# Autodesk Inventor assembly: Antriebsstrang
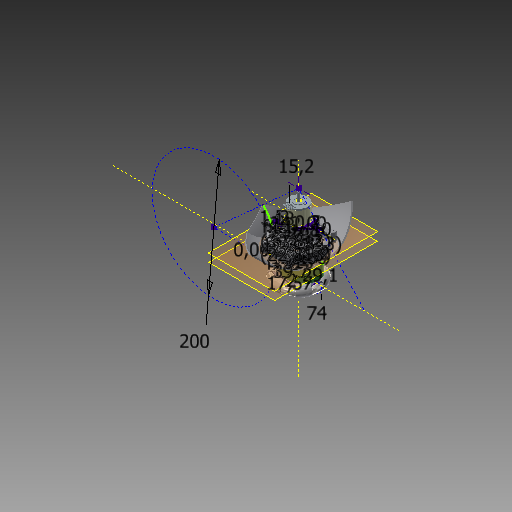
[picture p0: Inventor's stored thumbnail of the model, 512x512]
Saved by Autodesk Inventor 2018.3 (Build 223284000, 284)
## iProperties
Created: 2018-06-25
Part Number: Antriebsstrang
Material: Generisch
Document SubType Name: Assembly
Designer: JochenAlt
Author: JochenAlt
## Documents named in this file (15)
- D:\Projects\FlowerPot\CAD\DriveChain.iam
- D:\Projects\FlowerPot\CAD\OmniWheel.ipt
- D:\Projects\FlowerPot\CAD\Mounting Hub.ipt
- D:\Projects\FlowerPot\CAD\Encoder\Avago Encoder.iam
- D:\Projects\FlowerPot\CAD\HarmonicDrive-Axis.ipt
- C:\Users\JochenAlt\Documents\Inventor\Content Center Files\R2018\de-DE\AS 1420\AS 1420 - 1973 - M3 x 8.ipt
- C:\Users\JochenAlt\Documents\Inventor\Content Center Files\R2018\de-DE\DIN 912\DIN 912 - M2 x 0,4 x 8 x 7.ipt
- C:\Users\JochenAlt\Documents\Inventor\Content Center Files\R2018\de-DE\DIN 934\DIN 934 - M2 x 0,4.ipt
- D:\Projects\FlowerPot\CAD\BushOmniWheel.ipt
- C:\Users\JochenAlt\Documents\Inventor\Content Center Files\R2018\de-DE\DIN BEARING(1)\DIN 625 SKF - SKF 623.ipt
- D:\Projects\FlowerPot\CAD\Motor.iam
- D:\Projects\FlowerPot\CAD\PlanetaryGear\PlanetaryGear.iam
- D:\Projects\FlowerPot\CAD\BushingPlanetaryGearLeft.ipt
- D:\Projects\FlowerPot\CAD\DriveChainEnclosure.ipt
- D:\Projects\FlowerPot\CAD\EncoderBushRight.ipt
## Components (30 placed, 14 different names)
1. OmniWheel:1 — Passend:1, Passend:3, Passend:4, Passend:5, Passend:6, Passend:7, Passend:8, Passend:9, Passend:10, Passend:11, Passend:12, Passend:14, Passend:16, Passend:18, Passend:20, Passend:22, Passend:24
2. Mounting Hub:1 — Passend:1, Passend:25, Passend:30, Passend:31, Drehung:4, Drehung:5, Drehung:6
3. AS 1420 - Metrisch M3 x 8:1 — Passend:3, Passend:4
4. AS 1420 - Metrisch M3 x 8:2 — Passend:5, Passend:6, Passend:30
5. AS 1420 - Metrisch M3 x 8:3 — Passend:7, Passend:8
6. AS 1420 - Metrisch M3 x 8:4 — Passend:9, Passend:10
7. DIN 934 - ersetzt durch DIN EN 24032/28673/28674 M2:1 — Passend:13, Passend:14
8. DIN 934 - ersetzt durch DIN EN 24032/28673/28674 M2:2 — Passend:15, Passend:16
9. DIN 934 - ersetzt durch DIN EN 24032/28673/28674 M2:3 — Passend:17, Passend:18
10. DIN 934 - ersetzt durch DIN EN 24032/28673/28674 M2:4 — Passend:19, Passend:20
11. DIN 934 - ersetzt durch DIN EN 24032/28673/28674 M2:5 — Passend:21, Passend:22
12. DIN 934 - ersetzt durch DIN EN 24032/28673/28674 M2:6 — Passend:23, Passend:24
13. HarmonicDrive-Axis:2 — Passend:25, Passend:82, Passend:83, Passend:87, Passend:89, Passend:90, Drehung:4, Drehung:5, Drehung:6
14. BushOmniWheel:1 — Passend:31, Passend:83, Passend:84
15. DIN 625 SKF SKF 623:1 — Passend:80, Passend:81, Passend:82, Passend:84
16. DIN 625 SKF SKF 623:2 — Passend:79, Passend:85, Passend:86, Passend:91
17. Motor:1 [sub-assembly] — Passend:66, Passend:93, Passend:94
18. PlanetaryGear:1 [sub-assembly] — Passend:89, Passend:92, Passend:93, Passend:94
19. BushingPlanetaryGearLeft:2 — Passend:79
20. Avago Encoder:1 [sub-assembly] — Passend:87, Passend:88
21. DriveChainEnclosure:1 — Passend:80, Passend:81, Passend:85, Passend:86, Passend:88, Passend:95, Passend:96, Passend:97, Passend:98
22. EncoderBushRight:1 — Passend:90, Passend:91, Passend:92
23. DIN 912 - ersetzt durch DIN EN ISO 4762 M2 x 8:7 — Passend:95, Passend:96
24. DIN 912 - ersetzt durch DIN EN ISO 4762 M2 x 8:8 — Passend:97, Passend:98
25. DIN 912 - ersetzt durch DIN EN ISO 4762 M2 x 8:1 — Passend:11, Passend:12, Passend:13
26. DIN 912 - ersetzt durch DIN EN ISO 4762 M2 x 8:2 — Passend:23
27. DIN 912 - ersetzt durch DIN EN ISO 4762 M2 x 8:3 — Passend:21
28. DIN 912 - ersetzt durch DIN EN ISO 4762 M2 x 8:4 — Passend:19
29. DIN 912 - ersetzt durch DIN EN ISO 4762 M2 x 8:5 — Passend:17
30. DIN 912 - ersetzt durch DIN EN ISO 4762 M2 x 8:6 — Passend:15
## Component patterns: (6 elements, first: DIN 912 - ersetzt durch DIN EN ISO 4762 M2 x 8:1)
## Relationships (50: Mate 47, RelateRotation 3)
- Passend:1 [Mate]: OmniWheel:1 ↔ Mounting Hub:1
- Passend:3 [Mate]: OmniWheel:1 ↔ AS 1420 - Metrisch M3 x 8:1
- Passend:4 [Mate]: OmniWheel:1 ↔ AS 1420 - Metrisch M3 x 8:1
- Passend:5 [Mate]: OmniWheel:1 ↔ AS 1420 - Metrisch M3 x 8:2
- Passend:6 [Mate]: OmniWheel:1 ↔ AS 1420 - Metrisch M3 x 8:2
- Passend:7 [Mate]: OmniWheel:1 ↔ AS 1420 - Metrisch M3 x 8:3
- Passend:8 [Mate]: OmniWheel:1 ↔ AS 1420 - Metrisch M3 x 8:3
- Passend:9 [Mate]: OmniWheel:1 ↔ AS 1420 - Metrisch M3 x 8:4
- Passend:10 [Mate]: OmniWheel:1 ↔ AS 1420 - Metrisch M3 x 8:4
- Passend:11 [Mate]: OmniWheel:1 ↔ DIN 912 - ersetzt durch DIN EN ISO 4762 M2 x 8:1
- Passend:12 [Mate]: OmniWheel:1 ↔ DIN 912 - ersetzt durch DIN EN ISO 4762 M2 x 8:1
- Passend:13 [Mate]: DIN 934 - ersetzt durch DIN EN 24032/28673/28674 M2:1 ↔ DIN 912 - ersetzt durch DIN EN ISO 4762 M2 x 8:1
- Passend:14 [Mate]: OmniWheel:1 ↔ DIN 934 - ersetzt durch DIN EN 24032/28673/28674 M2:1
- Passend:15 [Mate]: DIN 934 - ersetzt durch DIN EN 24032/28673/28674 M2:2 ↔ DIN 912 - ersetzt durch DIN EN ISO 4762 M2 x 8:6
- Passend:16 [Mate]: OmniWheel:1 ↔ DIN 934 - ersetzt durch DIN EN 24032/28673/28674 M2:2
- Passend:17 [Mate]: DIN 934 - ersetzt durch DIN EN 24032/28673/28674 M2:3 ↔ DIN 912 - ersetzt durch DIN EN ISO 4762 M2 x 8:5
- Passend:18 [Mate]: OmniWheel:1 ↔ DIN 934 - ersetzt durch DIN EN 24032/28673/28674 M2:3
- Passend:19 [Mate]: DIN 934 - ersetzt durch DIN EN 24032/28673/28674 M2:4 ↔ DIN 912 - ersetzt durch DIN EN ISO 4762 M2 x 8:4
- Passend:20 [Mate]: OmniWheel:1 ↔ DIN 934 - ersetzt durch DIN EN 24032/28673/28674 M2:4
- Passend:21 [Mate]: DIN 934 - ersetzt durch DIN EN 24032/28673/28674 M2:5 ↔ DIN 912 - ersetzt durch DIN EN ISO 4762 M2 x 8:3
- Passend:22 [Mate]: OmniWheel:1 ↔ DIN 934 - ersetzt durch DIN EN 24032/28673/28674 M2:5
- Passend:23 [Mate]: DIN 934 - ersetzt durch DIN EN 24032/28673/28674 M2:6 ↔ DIN 912 - ersetzt durch DIN EN ISO 4762 M2 x 8:2
- Passend:24 [Mate]: OmniWheel:1 ↔ DIN 934 - ersetzt durch DIN EN 24032/28673/28674 M2:6
- Passend:25 [Mate]: Mounting Hub:1 ↔ HarmonicDrive-Axis:2
- Passend:30 [Mate]: Mounting Hub:1 ↔ AS 1420 - Metrisch M3 x 8:2
- Passend:31 [Mate]: Mounting Hub:1 ↔ BushOmniWheel:1
- Passend:66 [Mate]: Motor:1
- Passend:79 [Mate]: DIN 625 SKF SKF 623:2 ↔ BushingPlanetaryGearLeft:2
- Passend:80 [Mate]: DIN 625 SKF SKF 623:1 ↔ DriveChainEnclosure:1
- Passend:81 [Mate]: DIN 625 SKF SKF 623:1 ↔ DriveChainEnclosure:1
- Passend:82 [Mate]: HarmonicDrive-Axis:2 ↔ DIN 625 SKF SKF 623:1
- Passend:83 [Mate]: HarmonicDrive-Axis:2 ↔ BushOmniWheel:1
- Passend:84 [Mate]: BushOmniWheel:1 ↔ DIN 625 SKF SKF 623:1
- Passend:85 [Mate]: DIN 625 SKF SKF 623:2 ↔ DriveChainEnclosure:1
- Passend:86 [Mate]: DIN 625 SKF SKF 623:2 ↔ DriveChainEnclosure:1
- Passend:87 [Mate]: HarmonicDrive-Axis:2 ↔ Avago Encoder:1
- Passend:88 [Mate]: Avago Encoder:1 ↔ DriveChainEnclosure:1
- Passend:89 [Mate]: HarmonicDrive-Axis:2 ↔ PlanetaryGear:1
- Passend:90 [Mate]: HarmonicDrive-Axis:2 ↔ EncoderBushRight:1
- Passend:91 [Mate]: DIN 625 SKF SKF 623:2 ↔ EncoderBushRight:1
- Passend:92 [Mate]: PlanetaryGear:1 ↔ EncoderBushRight:1
- Passend:93 [Mate]: Motor:1 ↔ PlanetaryGear:1
- Passend:94 [Mate]: Motor:1 ↔ PlanetaryGear:1
- Drehung:4 [RelateRotation] (1 ul): Mounting Hub:1 ↔ HarmonicDrive-Axis:2
- Drehung:5 [RelateRotation] (1 ul): Mounting Hub:1 ↔ HarmonicDrive-Axis:2
- Drehung:6 [RelateRotation] (1 ul): Mounting Hub:1 ↔ HarmonicDrive-Axis:2
- Passend:95 [Mate]: DriveChainEnclosure:1 ↔ DIN 912 - ersetzt durch DIN EN ISO 4762 M2 x 8:7
- Passend:96 [Mate]: DriveChainEnclosure:1 ↔ DIN 912 - ersetzt durch DIN EN ISO 4762 M2 x 8:7
- Passend:97 [Mate]: DriveChainEnclosure:1 ↔ DIN 912 - ersetzt durch DIN EN ISO 4762 M2 x 8:8
- Passend:98 [Mate]: DriveChainEnclosure:1 ↔ DIN 912 - ersetzt durch DIN EN ISO 4762 M2 x 8:8
